# Autodesk Inventor assembly: złożenie czołg
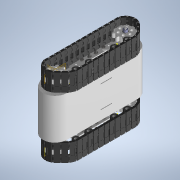
[picture p0: Inventor's stored thumbnail of the model, 180x180]
Saved by Autodesk Inventor 2021 (Build 250183000, 183)
## iProperties
Created: 2021-06-22
Part Number: złożenie czołg
Document SubType Name: Assembly
Designer: Łukasz
Author: Łukasz
## Documents named in this file (11)
- E:\GITHUB_Czołg\Szybki-Czolg-antyRadziecki\złożenie czołg.iam
- E:\GITHUB_Czołg\Szybki-Czolg-antyRadziecki\złożenie gąsienicy lewej.iam
- E:\GITHUB_Czołg\Szybki-Czolg-antyRadziecki\złożenie gąsienicy prawej.iam
- E:\GITHUB_Czołg\Szybki-Czolg-antyRadziecki\rama.ipt
- E:\GITHUB_Czołg\Szybki-Czolg-antyRadziecki\dystans na łożysk 6001 19mm.ipt
- E:\GITHUB_Czołg\Szybki-Czolg-antyRadziecki\blokada osi.ipt
- C:\Users\Łukasz\Documents\Inventor\Content Center Files\R2021\en-US\AS 1474(1)\AS 1474 - M8(1).ipt
- C:\Users\Łukasz\Documents\Inventor\Content Center Files\R2021\en-US\KS B 1002  C (2)\KS B 1002 - C  M 8 x 65(1).ipt
- C:\Users\Łukasz\Documents\Inventor\Content Center Files\R2021\en-US\BS 292 (I)\BS 292 Part 1 - 608 - 8 x 22 x 7.ipt
- C:\Users\Łukasz\Documents\Inventor\Content Center Files\R2021\en-US\AS 1237 (3.1)\AS 1237 - 8 mm(1)Aluminium-6061.ipt
- E:\GITHUB_Czołg\Szybki-Czolg-antyRadziecki\złożenie przekładni.iam
## Components (32 placed, 10 different names)
1. złożenie gąsienicy lewej:1 [sub-assembly] — Flush:2, Flush:3, Mate:1, Rotational:10, Rotational:11, Rigid:9, Rigid:10, Rigid:11, Rigid:12, Rigid:19, Angle:3
2. złożenie gąsienicy prawej:1 [sub-assembly] — Flush:2, Flush:3, Mate:1, Rotational:6, Rotational:7, Rigid:13, Rigid:14, Rigid:15, Rigid:16, Angle:1, Angle:2
3. AS 1237 (3.1) 8 mm - Aluminum 6061:1 — Rotational:5
4. AS 1237 (3.1) 8 mm - Aluminum 6061:2 — Rigid:18, Rigid:19
5. BS 292: Part 1 (I) (Metric) 608 - 8 x 22 x 7:4 — Rotational:2, Rotational:3, Rotational:5
6. BS 292: Part 1 (I) (Metric) 608 - 8 x 22 x 7:3 — Rotational:4
7. rama:1 — Rotational:2, Angle:1, Angle:2, Rigid:20, Angle:3, Rigid:21, Rigid:22, Rigid:23, Rigid:24, Mate:10, Mate:11
8. dystans na łożysk 6001 19mm:1 — Rotational:3, Rotational:4
9. blokada osi:1 — Rotational:6
10. blokada osi:2 — Rotational:7
11. dystans na łożysk 6001 19mm:2 — Rotational:8, Rotational:9
12. BS 292: Part 1 (I) (Metric) 608 - 8 x 22 x 7:2 — Rotational:9, Rigid:18, Rigid:20
13. BS 292: Part 1 (I) (Metric) 608 - 8 x 22 x 7:1 — Rotational:8
14. blokada osi:3 — Rotational:11
15. blokada osi:4 — Rotational:10
16. KS B 1002 C Regular Thread (Full Threaded) C  M 8 x 65:1
17. KS B 1002 C Regular Thread (Full Threaded) C  M 8 x 65:2
18. KS B 1002 C Regular Thread (Full Threaded) C  M 8 x 65:3
19. KS B 1002 C Regular Thread (Full Threaded) C  M 8 x 65:4
20. AS 1474 - Metric M8:1 — Rigid:21
21. AS 1474 - Metric M8:2 — Rigid:16
22. AS 1474 - Metric M8:3 — Rigid:11
23. AS 1474 - Metric M8:4 — Rigid:15
24. AS 1474 - Metric M8:5 — Rigid:13
25. AS 1474 - Metric M8:6 — Rigid:12
26. AS 1474 - Metric M8:7 — Rigid:22
27. AS 1474 - Metric M8:8 — Rigid:14
28. AS 1474 - Metric M8:9 — Rigid:9
29. AS 1474 - Metric M8:10 — Rigid:10
30. AS 1474 - Metric M8:11 — Rigid:23
31. AS 1474 - Metric M8:12 — Rigid:24
32. złożenie przekładni:2 [sub-assembly] — Mate:10, Mate:11
## Relationships (33: WeldJoint 15, RevoluteJoint 10, Mate 3, Angle 3, Flush 2)
- Flush:2: złożenie gąsienicy lewej:1 ↔ złożenie gąsienicy prawej:1
- Flush:3: złożenie gąsienicy lewej:1 ↔ złożenie gąsienicy prawej:1
- Mate:1 (200 mm): złożenie gąsienicy lewej:1 ↔ złożenie gąsienicy prawej:1
- Rotational:2 [RevoluteJoint]: BS 292: Part 1 (I) (Metric) 608 - 8 x 22 x 7:4 ↔ rama:1
- Rotational:3 [RevoluteJoint]: BS 292: Part 1 (I) (Metric) 608 - 8 x 22 x 7:4 ↔ dystans na łożysk 6001 19mm:1
- Rotational:4 [RevoluteJoint]: BS 292: Part 1 (I) (Metric) 608 - 8 x 22 x 7:3 ↔ dystans na łożysk 6001 19mm:1
- Rotational:5 [RevoluteJoint]: AS 1237 (3.1) 8 mm - Aluminum 6061:1 ↔ BS 292: Part 1 (I) (Metric) 608 - 8 x 22 x 7:4
- Rotational:6 [RevoluteJoint]: złożenie gąsienicy prawej:1 ↔ blokada osi:1
- Rotational:7 [RevoluteJoint]: złożenie gąsienicy prawej:1 ↔ blokada osi:2
- Rotational:8 [RevoluteJoint]: dystans na łożysk 6001 19mm:2 ↔ BS 292: Part 1 (I) (Metric) 608 - 8 x 22 x 7:1
- Rotational:9 [RevoluteJoint]: dystans na łożysk 6001 19mm:2 ↔ BS 292: Part 1 (I) (Metric) 608 - 8 x 22 x 7:2
- Rotational:10 [RevoluteJoint]: złożenie gąsienicy lewej:1 ↔ blokada osi:4
- Rotational:11 [RevoluteJoint]: złożenie gąsienicy lewej:1 ↔ blokada osi:3
- Rigid:9 [WeldJoint]: złożenie gąsienicy lewej:1 ↔ AS 1474 - Metric M8:9
- Rigid:10 [WeldJoint]: złożenie gąsienicy lewej:1 ↔ AS 1474 - Metric M8:10
- Rigid:11 [WeldJoint]: złożenie gąsienicy lewej:1 ↔ AS 1474 - Metric M8:3
- Rigid:12 [WeldJoint]: złożenie gąsienicy lewej:1 ↔ AS 1474 - Metric M8:6
- Rigid:13 [WeldJoint]: złożenie gąsienicy prawej:1 ↔ AS 1474 - Metric M8:5
- Rigid:14 [WeldJoint]: złożenie gąsienicy prawej:1 ↔ AS 1474 - Metric M8:8
- Rigid:15 [WeldJoint]: złożenie gąsienicy prawej:1 ↔ AS 1474 - Metric M8:4
- Rigid:16 [WeldJoint]: złożenie gąsienicy prawej:1 ↔ AS 1474 - Metric M8:2
- Angle:1 (0 deg): złożenie gąsienicy prawej:1 ↔ rama:1
- Angle:2 (0 deg): złożenie gąsienicy prawej:1 ↔ rama:1
- Rigid:18 [WeldJoint]: AS 1237 (3.1) 8 mm - Aluminum 6061:2 ↔ BS 292: Part 1 (I) (Metric) 608 - 8 x 22 x 7:2
- Rigid:19 [WeldJoint]: złożenie gąsienicy lewej:1 ↔ AS 1237 (3.1) 8 mm - Aluminum 6061:2
- Rigid:20 [WeldJoint]: rama:1 ↔ BS 292: Part 1 (I) (Metric) 608 - 8 x 22 x 7:2
- Angle:3 (0 deg): złożenie gąsienicy lewej:1 ↔ rama:1
- Rigid:21 [WeldJoint]: rama:1 ↔ AS 1474 - Metric M8:1
- Rigid:22 [WeldJoint]: rama:1 ↔ AS 1474 - Metric M8:7
- Rigid:23 [WeldJoint]: rama:1 ↔ AS 1474 - Metric M8:11
- Rigid:24 [WeldJoint]: rama:1 ↔ AS 1474 - Metric M8:12
- Mate:10: rama:1 ↔ złożenie przekładni:2
- Mate:11: rama:1 ↔ złożenie przekładni:2
